# Autodesk Inventor assembly: ServiceRoboter
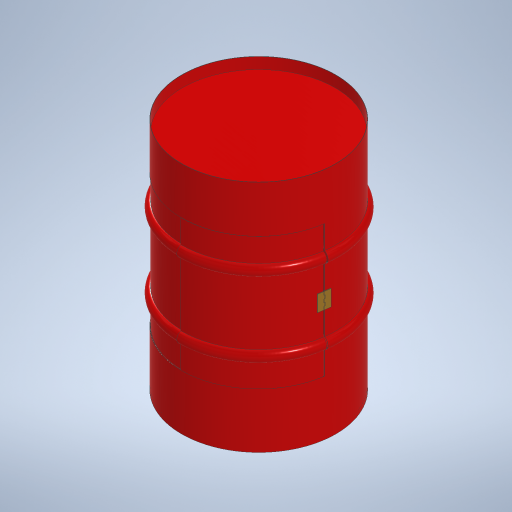
[picture p0: Inventor's stored thumbnail of the model, 512x512]
Saved by Autodesk Inventor 2024 (Build 280153000, 153)
## iProperties
Created: 2023-11-30
Part Number: ServiceRoboter
Document SubType Name: Assembly
Designer: Daniel Nussbaum
Author: Daniel Nussbaum
## Documents named in this file (8)
- C:\GitHubDesktop\3d-model\service_roboter\ServiceRoboter.iam
- C:\GitHubDesktop\3d-model\service_roboter\Fass.ipt
- C:\GitHubDesktop\3d-model\service_roboter\FassTuer.ipt
- C:\GitHubDesktop\3d-model\service_roboter\SchnierTeilA.ipt
- C:\GitHubDesktop\3d-model\service_roboter\SchanierTeilB.ipt
- C:\GitHubDesktop\3d-model\service_roboter\SchnierTeilA_CPY.ipt
- C:\GitHubDesktop\3d-model\service_roboter\SchanierTeilB_CPY.ipt
- C:\GitHubDesktop\3d-model\basis_roboter\Deckel.ipt
## Components (8 placed, 7 different names)
1. Fass:1 — Rigid:1, Rigid:2, Rigid:5
2. FassTuer:1 — Rigid:3
3. FassTuer:2 — Rigid:4
4. SchnierTeilA:1 — Rotational:1, Rigid:1
5. SchanierTeilB:1 — Rotational:1, Rigid:4
6. SchnierTeilA_CPY:1 — Rotational:2, Rigid:2
7. SchanierTeilB_CPY:1 — Rotational:2, Rigid:3
8. Deckel:1 — Rigid:5
## Relationships (7: WeldJoint 5, RevoluteJoint 2)
- Rotational:1 [RevoluteJoint]: SchnierTeilA:1 ↔ SchanierTeilB:1
- Rotational:2 [RevoluteJoint]: SchnierTeilA_CPY:1 ↔ SchanierTeilB_CPY:1
- Rigid:1 [WeldJoint]: Fass:1 ↔ SchnierTeilA:1
- Rigid:2 [WeldJoint]: Fass:1 ↔ SchnierTeilA_CPY:1
- Rigid:3 [WeldJoint]: FassTuer:1 ↔ SchanierTeilB_CPY:1
- Rigid:4 [WeldJoint]: FassTuer:2 ↔ SchanierTeilB:1
- Rigid:5 [WeldJoint] (-40 mm): Fass:1 ↔ Deckel:1
